# Autodesk Inventor assembly: Shooter Assembly
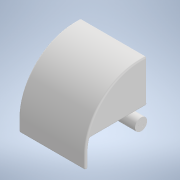
[picture p0: Inventor's stored thumbnail of the model, 180x180]
Saved by Autodesk Inventor 2020 (Build 240168000, 168)
## iProperties
Created: 2020-01-14
Part Number: Shooter Assembly
Document SubType Name: Assembly
Designer: woodn
Author: woodn
## Documents named in this file (5)
- C:\Users\woodn\3D Objects\Shooter Assembly.iam
- C:\Users\woodn\3D Objects\Shooter shell.ipt
- C:\Users\woodn\3D Objects\FRC Ball.ipt
- C:\Users\woodn\3D Objects\pin.ipt
- C:\Users\woodn\3D Objects\Compliance wheel.ipt
## Components (4 placed, 4 different names)
1. Shooter shell:1 — Mate:1, Mate:3, Flush:1, Mate:4, Mate:6, Mate:7
2. pin:1 — Mate:1, Flush:1, Mate:4, Mate:5, Mate:7, Mate:8
3. Compliance wheel:1 — Mate:3, Mate:5, Mate:6, Mate:8, Transitional:1
4. FRC Ball:1 — Transitional:1
## Relationships (9: Mate 7, Flush 1, Transitional 1)
- Mate:1: Shooter shell:1 ↔ pin:1
- Mate:3: Shooter shell:1 ↔ Compliance wheel:1
- Flush:1: Shooter shell:1 ↔ pin:1
- Mate:4: Shooter shell:1 ↔ pin:1
- Mate:5: pin:1 ↔ Compliance wheel:1
- Mate:6: Shooter shell:1 ↔ Compliance wheel:1
- Mate:7: Shooter shell:1 ↔ pin:1
- Mate:8: pin:1 ↔ Compliance wheel:1
- Transitional:1: Compliance wheel:1 ↔ FRC Ball:1
